# Autodesk Inventor assembly: Bildverarbeitungsband_Blech
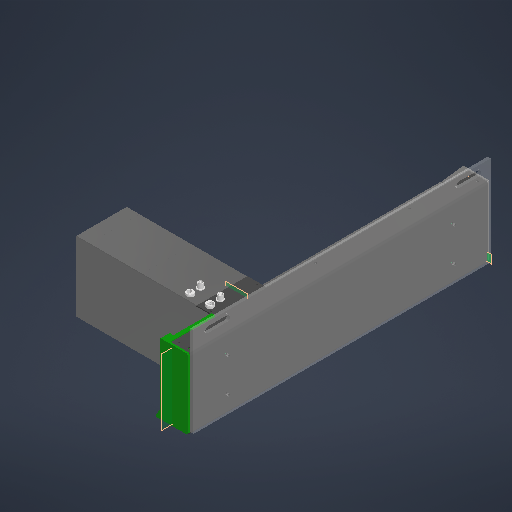
[picture p0: Inventor's stored thumbnail of the model, 512x512]
Saved by Autodesk Inventor 2026.1 (Build 301233020, 233B)
## iProperties
Created: 2025-04-28
Part Number: Bildverarbeitungsband_Blech
Document SubType Name: Assembly
Designer: iopeter
Author: iopeter
## Documents named in this file (16)
- C:\Users\neume\Desktop\MCI\Robotik_Projekt\Optimierung-Laboraufgabe-Robotik\Abgabe_Optimierung_Robotik\Konstruktion\Inventor_ConveyorTracking\Bildverarbeitungsband_Blech.iam
- C:\Users\neume\Desktop\MCI\Robotik_Projekt\Optimierung-Laboraufgabe-Robotik\Abgabe_Optimierung_Robotik\Konstruktion\Inventor_ConveyorTracking\FR-40-160-800-K.ipt
- C:\Users\neume\Desktop\MCI\Robotik_Projekt\Optimierung-Laboraufgabe-Robotik\Abgabe_Optimierung_Robotik\Konstruktion\Inventor_ConveyorTracking\U-Blech-Bild.ipt
- C:\Users\neume\Desktop\MCI\Robotik_Projekt\Optimierung-Laboraufgabe-Robotik\Abgabe_Optimierung_Robotik\Konstruktion\Inventor_ConveyorTracking\Harting_Flansch_V1.ipt
- C:\Users\neume\Desktop\MCI\Robotik_Projekt\Optimierung-Laboraufgabe-Robotik\Abgabe_Optimierung_Robotik\Konstruktion\Inventor_ConveyorTracking\ethernet_coupler.ipt
- C:\Users\neume\Desktop\MCI\Robotik_Projekt\Optimierung-Laboraufgabe-Robotik\Abgabe_Optimierung_Robotik\Konstruktion\Inventor_ConveyorTracking\1747871.ipt
- C:\Users\neume\Desktop\MCI\Robotik_Projekt\Optimierung-Laboraufgabe-Robotik\Abgabe_Optimierung_Robotik\Konstruktion\Inventor_ConveyorTracking\Kameraturm.ipt
- C:\Users\neume\Desktop\MCI\Robotik_Projekt\Optimierung-Laboraufgabe-Robotik\Abgabe_Optimierung_Robotik\Konstruktion\Inventor_ConveyorTracking\In-Sight 2800 Multi Torch Straight.ipt
- C:\Users\neume\Desktop\MCI\Robotik_Projekt\Optimierung-Laboraufgabe-Robotik\Abgabe_Optimierung_Robotik\Konstruktion\Inventor_ConveyorTracking\Kameraturm_Deckel.ipt
- C:\Users\neume\Desktop\MCI\Robotik_Projekt\Optimierung-Laboraufgabe-Robotik\Abgabe_Optimierung_Robotik\Konstruktion\Inventor_ConveyorTracking\Plexi_Bildverarbeitungsband.ipt
- C:\Users\neume\Desktop\MCI\Robotik_Projekt\Optimierung-Laboraufgabe-Robotik\Abgabe_Optimierung_Robotik\Konstruktion\Inventor_ConveyorTracking\Kameraturm_Abdeckung_Unten.ipt
- C:\Users\neume\Desktop\MCI\Robotik_Projekt\Optimierung-Laboraufgabe-Robotik\Abgabe_Optimierung_Robotik\Konstruktion\Inventor_ConveyorTracking\Kameraturm_Cognex_Halter.ipt
- C:\Users\neume\Desktop\MCI\Robotik_Projekt\Optimierung-Laboraufgabe-Robotik\Abgabe_Optimierung_Robotik\Konstruktion\Inventor_ConveyorTracking\Endstueck_cnv_new.ipt
- C:\Users\neume\Desktop\MCI\Robotik_Projekt\Optimierung-Laboraufgabe-Robotik\Abgabe_Optimierung_Robotik\Konstruktion\Inventor_ConveyorTracking\Conveyor_Bundbauteil_new.ipt
- C:\Users\neume\Desktop\MCI\Robotik_Projekt\Optimierung-Laboraufgabe-Robotik\Abgabe_Optimierung_Robotik\Konstruktion\Inventor_ConveyorTracking\Kameraturm_Base_V3.ipt
- C:\Users\neume\Desktop\MCI\Robotik_Projekt\Optimierung-Laboraufgabe-Robotik\Abgabe_Optimierung_Robotik\Konstruktion\Inventor_ConveyorTracking\cnv_endstueck_V2.ipt
## Components (17 placed, 16 different names)
1. FR-40-160-800-K:1 — Fluchtend:1, Fluchtend:6, Passend:2
2. U-Blech-Bild:1 — Fluchtend:1, Passend:1, Fluchtend:6, Passend:2, Passend:3, Fluchtend:7, Passend:4, Passend:5, Fluchtend:14, Passend:12, Passend:13, Passend:14, Passend:15, Passend:17
3. Harting_Flansch_V1:1 — Passend:3, Fluchtend:7, Passend:4
4. ethernet_coupler:1 — Passend:1
5. M12_F_Panelmount — Passend:5
6. Plexi_Bildverarbeitungsband:1 — Fluchtend:14
7. Kameraturm_Cognex_Halter:1 — Fluchtend:22
8. Endstueck_cnv_new:1 — Passend:12
9. Conveyor_Bundbauteil_new:1 — Passend:13
10. Kameraturm_Base_V3:1 — Passend:14, Passend:15
11. cnv_endstueck_noHarting — Passend:17
12. Kameraturm_Abdeckung_Unten:1 — Fluchtend:20, Fluchtend:21
13. Kameraturm:1 — Fluchtend:13, Passend:7, Passend:9, Fluchtend:20, Fluchtend:21, Fluchtend:22
14. In-Sight 2800 Multi Torch Straight:1
15. Kameraturm_Deckel:1 — Fluchtend:13
16. ethernet_coupler:2 — Passend:7
17. 1747871:2 — Passend:9
## Relationships (20: Mate 12, Flush 8)
- Fluchtend:1 [Flush] (10 mm): FR-40-160-800-K:1 ↔ U-Blech-Bild:1
- Passend:1 [Mate]: U-Blech-Bild:1 ↔ ethernet_coupler:1
- Fluchtend:6 [Flush] (192 mm): FR-40-160-800-K:1 ↔ U-Blech-Bild:1
- Passend:2 [Mate]: FR-40-160-800-K:1 ↔ U-Blech-Bild:1
- Passend:3 [Mate]: U-Blech-Bild:1 ↔ Harting_Flansch_V1:1
- Fluchtend:7 [Flush]: U-Blech-Bild:1 ↔ Harting_Flansch_V1:1
- Passend:4 [Mate]: U-Blech-Bild:1 ↔ Harting_Flansch_V1:1
- Passend:5 [Mate]: U-Blech-Bild:1 ↔ M12_F_Panelmount
- Fluchtend:13 [Flush]: Kameraturm:1 ↔ Kameraturm_Deckel:1
- Passend:7 [Mate]: Kameraturm:1 ↔ ethernet_coupler:2
- Fluchtend:14 [Flush]: U-Blech-Bild:1 ↔ Plexi_Bildverarbeitungsband:1
- Passend:9 [Mate]: Kameraturm:1 ↔ 1747871:2
- Fluchtend:20 [Flush]: Kameraturm_Abdeckung_Unten:1 ↔ Kameraturm:1
- Fluchtend:21 [Flush]: Kameraturm_Abdeckung_Unten:1 ↔ Kameraturm:1
- Fluchtend:22 [Flush]: Kameraturm_Cognex_Halter:1 ↔ Kameraturm:1
- Passend:12 [Mate]: U-Blech-Bild:1 ↔ Endstueck_cnv_new:1
- Passend:13 [Mate]: U-Blech-Bild:1 ↔ Conveyor_Bundbauteil_new:1
- Passend:14 [Mate]: U-Blech-Bild:1 ↔ Kameraturm_Base_V3:1
- Passend:15 [Mate]: U-Blech-Bild:1 ↔ Kameraturm_Base_V3:1
- Passend:17 [Mate]: U-Blech-Bild:1 ↔ cnv_endstueck_noHarting
